# Autodesk Inventor assembly: catapult assembly new arm
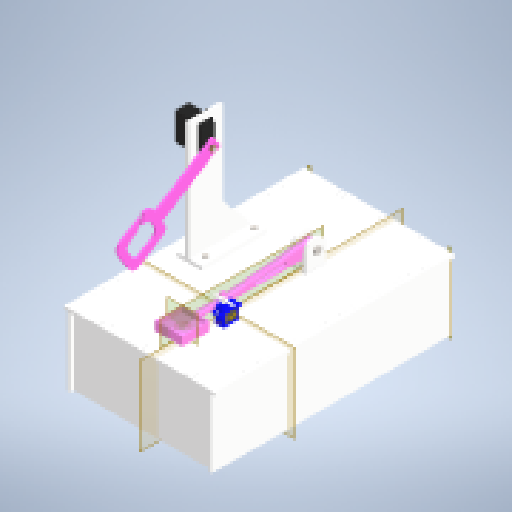
[picture p0: Inventor's stored thumbnail of the model, 512x512]
Saved by Autodesk Inventor 2025.3 (Build 293356000, 356)
## iProperties
Created: 2026-04-16
Part Number: catapult assembly new arm
Description: STEP AP214
Document SubType Name: Assembly
Designer: logien
Sending System: SolidWorks 2022
Preprocessor: SwSTEP 2.0
Title: catapult assembly new arm.STEP
Revision Number: ANY
## Documents named in this file (16)
- C:\Users\logys\OneDrive\Desktop\ASU\Spring 2026\Basics of mechatronics\project\catapult assembly new arm.iam
- C:\Users\logys\OneDrive\Desktop\ASU\Spring 2026\Basics of mechatronics\project\catapult assembly new arm\catapult assembly new arm\Base.ipt
- C:\Users\logys\OneDrive\Desktop\ASU\Spring 2026\Basics of mechatronics\project\catapult assembly new arm\catapult assembly new arm\arm holder.ipt
- C:\Users\logys\OneDrive\Desktop\ASU\Spring 2026\Basics of mechatronics\project\catapult assembly new arm\catapult assembly new arm\Catapult arm.ipt
- C:\Users\logys\OneDrive\Desktop\ASU\Spring 2026\Basics of mechatronics\project\catapult assembly new arm\catapult assembly new arm\mount.ipt
- C:\Users\logys\OneDrive\Desktop\ASU\Spring 2026\Basics of mechatronics\project\catapult assembly new arm\catapult assembly new arm\loader.ipt
- C:\Users\logys\OneDrive\Desktop\ASU\Spring 2026\Basics of mechatronics\project\catapult assembly new arm\catapult assembly new arm\servo 1 assembly.iam
- C:\Users\logys\OneDrive\Desktop\ASU\Spring 2026\Basics of mechatronics\project\catapult assembly new arm\catapult assembly new arm\plain washer normal grade a_iso_Washer ISO 7089 - 6.ipt
- C:\Users\logys\OneDrive\Desktop\ASU\Spring 2026\Basics of mechatronics\project\catapult assembly new arm\catapult assembly new arm\hex nut style 1 gradeab_iso_ISO - 4032 - M6 - W - N.ipt
- C:\Users\logys\OneDrive\Desktop\ASU\Spring 2026\Basics of mechatronics\project\catapult assembly new arm\catapult assembly new arm\hex bolt gradeab_iso_ISO 4014 - M6 x 30 x 18-N.ipt
- C:\Users\logys\OneDrive\Desktop\ASU\Spring 2026\Basics of mechatronics\project\catapult assembly new arm\catapult assembly new arm\hex nut style 1 gradeab_iso_ISO - 4032 - M4 - W - N.ipt
- C:\Users\logys\OneDrive\Desktop\ASU\Spring 2026\Basics of mechatronics\project\catapult assembly new arm\catapult assembly new arm\hex screw gradeab_iso_ISO 4017 - M4 x 16-N.ipt
- C:\Users\logys\OneDrive\Desktop\ASU\Spring 2026\Basics of mechatronics\project\catapult assembly new arm\catapult assembly new arm\Servo MG996R_Predeterminado.ipt
- C:\Users\logys\OneDrive\Desktop\ASU\Spring 2026\Basics of mechatronics\project\catapult assembly new arm\catapult assembly new arm\[4145] TowerPro SG90 Mini Servo-SunRobotics_in-Pt5_BS EN ISO 7045 - M2 x 8 - Z .ipt
- C:\Users\logys\OneDrive\Desktop\ASU\Spring 2026\Basics of mechatronics\project\catapult assembly new arm\catapult assembly new arm\width.ipt
- C:\Users\logys\OneDrive\Desktop\ASU\Spring 2026\Basics of mechatronics\project\catapult assembly new arm\catapult assembly new arm\length.ipt
## Components (28 placed, 28 different names)
1. Base_1 — Mate:1, Mate:4, Mate:6, Mate:7, Mate:8, Mate:9, Mate:10, Mate:11, Mate:12, Mate:13, Mate:14, Mate:17, Mate:18, Mate:19, Mate:20, Insert:12, Insert:13, Insert:14, Insert:15, Insert:16, Mate:25
2. arm holder_2 — Mate:1, Insert:1, Insert:2, Insert:3, Insert:4, Insert:7, Insert:8, Mate:19, Mate:20
3. Catapult arm_3 — Mate:3, Insert:6
4. mount_4 — Mate:12, Insert:5, Mate:13, Mate:14, Mate:15, Mate:16, Mate:21, Mate:22, Mate:23, Mate:24, Insert:11, Insert:17, Insert:18
5. loader_5 — Insert:9
6. servo 1 assembly_6 [sub-assembly] — Mate:4, Mate:5, Mate:26
7. plain washer normal grade a_iso_Washer ISO 7089 - 6_7 — Insert:8
8. plain washer normal grade a_iso_Washer ISO 7089 - 6_8 — Insert:6, Insert:7
9. hex nut style 1 gradeab_iso_ISO - 4032 - M6 - W - N_9 — Insert:2
10. hex bolt gradeab_iso_ISO 4014 - M6 x 30 x 18-N_10 — Insert:1, Mate:3
11. hex nut style 1 gradeab_iso_ISO - 4032 - M4 - W - N_11 — Insert:16
12. hex nut style 1 gradeab_iso_ISO - 4032 - M4 - W - N_12 — Mate:25
13. hex screw gradeab_iso_ISO 4017 - M4 x 16-N_13 — Insert:4
14. hex screw gradeab_iso_ISO 4017 - M4 x 16-N_14 — Insert:3
15. Servo MG996R_Predeterminado_15 — Mate:21, Mate:22, Mate:23, Mate:24, Insert:9, Insert:10
16. [4145] TowerPro SG90 Mini Servo-SunRobotics_in-Pt5_BS EN ISO 7045 - M2 x 8 - Z - 8S_16 — Insert:10
17. hex screw gradeab_iso_ISO 4017 - M4 x 16-N_17 — Insert:11
18. hex screw gradeab_iso_ISO 4017 - M4 x 16-N_18 — Insert:5
19. hex screw gradeab_iso_ISO 4017 - M4 x 16-N_19 — Mate:16, Insert:18
20. hex screw gradeab_iso_ISO 4017 - M4 x 16-N_20 — Mate:15, Insert:17
21. hex nut style 1 gradeab_iso_ISO - 4032 - M4 - W - N_21 — Insert:12
22. hex nut style 1 gradeab_iso_ISO - 4032 - M4 - W - N_22 — Insert:15
23. hex nut style 1 gradeab_iso_ISO - 4032 - M4 - W - N_23 — Insert:13
24. hex nut style 1 gradeab_iso_ISO - 4032 - M4 - W - N_24 — Insert:14
25. width_25 — Mate:8, Mate:9, Flush:2
26. length_26 — Mate:10, Mate:11
27. length_27 — Flush:1, Mate:6, Mate:7
28. width_28 — Mate:17, Mate:18
## Relationships (45: Mate 25, Insert 18, Flush 2)
- Mate:1: Base_1 ↔ arm holder_2
- Insert:1: arm holder_2 ↔ hex bolt gradeab_iso_ISO 4014 - M6 x 30 x 18-N_10
- Insert:2: arm holder_2 ↔ hex nut style 1 gradeab_iso_ISO - 4032 - M6 - W - N_9
- Insert:3: arm holder_2 ↔ hex screw gradeab_iso_ISO 4017 - M4 x 16-N_14
- Insert:4: arm holder_2 ↔ hex screw gradeab_iso_ISO 4017 - M4 x 16-N_13
- Mate:3: Catapult arm_3 ↔ hex bolt gradeab_iso_ISO 4014 - M6 x 30 x 18-N_10
- Mate:4: Base_1 ↔ servo 1 assembly_6
- Flush:1 (-82 mm): length_27
- Mate:5: servo 1 assembly_6
- Mate:6: Base_1 ↔ length_27
- Mate:7: Base_1 ↔ length_27
- Mate:8: Base_1 ↔ width_25
- Mate:9: Base_1 ↔ width_25
- Mate:10: Base_1 ↔ length_26
- Mate:11: Base_1 ↔ length_26
- Mate:12: Base_1 ↔ mount_4
- Insert:5: mount_4 ↔ hex screw gradeab_iso_ISO 4017 - M4 x 16-N_18
- Mate:13: Base_1 ↔ mount_4
- Mate:14: Base_1 ↔ mount_4
- Mate:15: mount_4 ↔ hex screw gradeab_iso_ISO 4017 - M4 x 16-N_20
- Mate:16: mount_4 ↔ hex screw gradeab_iso_ISO 4017 - M4 x 16-N_19
- Mate:17: Base_1 ↔ width_28
- Mate:18: Base_1 ↔ width_28
- Insert:6: Catapult arm_3 ↔ plain washer normal grade a_iso_Washer ISO 7089 - 6_8
- Insert:7: arm holder_2 ↔ plain washer normal grade a_iso_Washer ISO 7089 - 6_8
- Insert:8: arm holder_2 ↔ plain washer normal grade a_iso_Washer ISO 7089 - 6_7
- Mate:19: Base_1 ↔ arm holder_2
- Mate:20: Base_1 ↔ arm holder_2
- Mate:21: mount_4 ↔ Servo MG996R_Predeterminado_15
- Mate:22: mount_4 ↔ Servo MG996R_Predeterminado_15
- Mate:23: mount_4 ↔ Servo MG996R_Predeterminado_15
- Mate:24: mount_4 ↔ Servo MG996R_Predeterminado_15
- Insert:9: loader_5 ↔ Servo MG996R_Predeterminado_15
- Insert:10: Servo MG996R_Predeterminado_15 ↔ [4145] TowerPro SG90 Mini Servo-SunRobotics_in-Pt5_BS EN ISO 7045 - M2 x 8 - Z - 8S_16
- Insert:11: mount_4 ↔ hex screw gradeab_iso_ISO 4017 - M4 x 16-N_17
- Insert:12: Base_1 ↔ hex nut style 1 gradeab_iso_ISO - 4032 - M4 - W - N_21
- Insert:13: Base_1 ↔ hex nut style 1 gradeab_iso_ISO - 4032 - M4 - W - N_23
- Insert:14: Base_1 ↔ hex nut style 1 gradeab_iso_ISO - 4032 - M4 - W - N_24
- Insert:15: Base_1 ↔ hex nut style 1 gradeab_iso_ISO - 4032 - M4 - W - N_22
- Insert:16: Base_1 ↔ hex nut style 1 gradeab_iso_ISO - 4032 - M4 - W - N_11
- Mate:25: Base_1 ↔ hex nut style 1 gradeab_iso_ISO - 4032 - M4 - W - N_12
- Insert:17: mount_4 ↔ hex screw gradeab_iso_ISO 4017 - M4 x 16-N_20
- Insert:18: mount_4 ↔ hex screw gradeab_iso_ISO 4017 - M4 x 16-N_19
- Flush:2 (-105 mm): width_25
- Mate:26: servo 1 assembly_6
